# Autodesk Inventor assembly: Assembly_v1
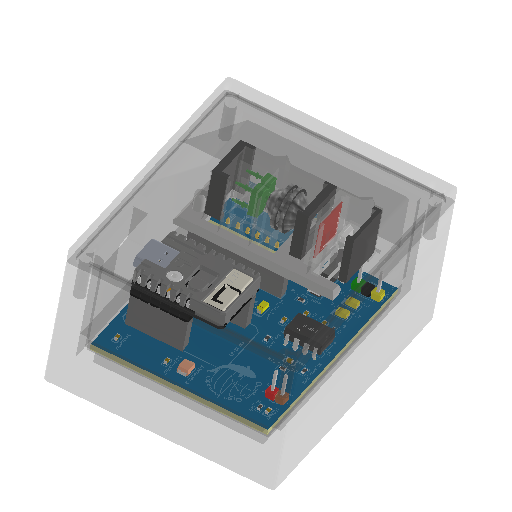
[picture p0: Inventor's stored thumbnail of the model, 512x512]
Saved by Autodesk Inventor 2026.1 (Build 301233020, 233B)
## iProperties
Created: 2026-01-21
Part Number: Assembly_v1
Document SubType Name: Assembly
Designer: samuel
Author: samuel
## Documents named in this file (18)
- E:\Fraunhofer\Design\Assembly_Box.iam
- E:\Fraunhofer\Design\Box_bottom_v2.ipt
- E:\Fraunhofer\Design\Parts\ads1015 ads1115 module type1\ads1015 ads1115 module type1\ads1015 ads1115 module type1.ipt
- E:\Fraunhofer\Design\Parts\USB C Male connector cable\USB C Male connector cable\USB C Male connector cable.ipt
- E:\Fraunhofer\Design\Assembly_NV__Optical_Modules.iam
- E:\Fraunhofer\Design\Parts\3D_PCB5_2026-02-13\3D_PCB5_2026-02-13\ESP32-S3~M5Stack StampS3 ~M5STAMP-S3.step~11hL.iam
- E:\Fraunhofer\Design\Parts\female-header-pins-2.snapshot.2\Female 6 Pin Header_\Female 6 Pin Header_\Female 6 Pin Header_.ipt
- E:\Fraunhofer\Design\Parts\female-header-pins-2.snapshot.2\Female 10 Pin Header\Female 10 Pin Header\Female 10 Pin Header.ipt
- E:\Fraunhofer\Design\Parts\female-header-pins-2.snapshot.2\Female 9 Pin Header\Female 9 Pin Header\Female 9 Pin Header.ipt
- E:\Fraunhofer\Design\Parts\3D_PCB5\3D_PCB5\3D_PCB5.iam
- E:\Fraunhofer\Design\Parts\2-54mm-male-pin-header-1.snapshot.3\Step\100mill Male Pin Header_10P_Y\100mill Male Pin Header_6P_Bk\100mill Male Pin Header_6P_Bk.ipt
- E:\Fraunhofer\Design\Parts\2-54mm-male-pin-header-1.snapshot.3\Step\100mill Male Pin Header_10P_Y\100mill Male Pin Header_9P_Bk\100mill Male Pin Header_9P_Bk.ipt
- E:\Fraunhofer\Design\Parts\2-54mm-male-pin-header-1.snapshot.3\Step\100mill Male Pin Header_2P_Bk\100mill Male Pin Header_2P_Bk\100mill Male Pin Header_2P_Bk.ipt
- E:\Fraunhofer\Design\Parts\2-54mm-male-pin-header-1.snapshot.3\Step\100mill Male Pin Header_3P_Bk\100mill Male Pin Header_3P_Bk\100mill Male Pin Header_3P_Bk.ipt
- E:\Fraunhofer\Design\Parts\dupont-jumper-wire-1.snapshot.3\Dupont Jumper Wire F-F\Dupont Jumper Wire F-F\Dupont Jumper Wire F-F.ipt
- E:\Fraunhofer\Design\Parts\dupont-jumper-wire-1.snapshot.3\Dupont Jumper Wire F-F\Dupont Jumper Wire F-F\Dupont Jumper Wire F-F - yellow.ipt
- E:\Fraunhofer\Design\Parts\dupont-jumper-wire-1.snapshot.3\Dupont Jumper Wire F-F\Dupont Jumper Wire F-F\Dupont Jumper Wire F-F - green.ipt
- E:\Fraunhofer\Design\Parts\dupont-jumper-wire-1.snapshot.3\Dupont Jumper Wire F-F\Dupont Jumper Wire F-F\Dupont Jumper Wire F-F - black.ipt
## Components (17 placed, 17 different names)
1. Box_bottom_v2:1 — Mate:10, Mate:13, Mate:21, Flush:19, Flush:20
2. ads1015 ads1115 module type1:1 — Flush:6, Flush:7, Mate:4
3. USB C Male connector cable:1 — Mate:19, Mate:20
4. Assembly_NV__Optical_Modules:1 [sub-assembly] — Flush:19, Flush:20
5. ESP32-S3~M5Stack StampS3 ~M5STAMP-S3.step~11hL:1 [sub-assembly] — Mate:8, Flush:8, Flush:9, Mate:9, Flush:10, Flush:11, Mate:19, Mate:20
6. 100mill Male Pin Header_6P_Bk:1 — Flush:12, Flush:13
7. 100mill Male Pin Header_9P_Bk:1 — Flush:14, Flush:15
8. Female 6 Pin Header_:1 — Mate:8, Flush:8, Flush:9, Mate:14, Mate:15, Mate:18, Flush:12, Flush:13
9. Female 10 Pin Header:1 — Flush:6, Flush:7, Mate:4, Mate:12, Mate:16, Mate:17
10. Female 9 Pin Header:1 — Mate:9, Flush:10, Flush:11, Flush:14, Flush:15
11. 3D_PCB5:1 [sub-assembly] — Mate:10, Mate:12, Mate:13, Mate:14, Mate:15, Mate:16, Mate:17, Mate:18, Mate:21, Mate:22, Flush:16, Mate:23, Flush:17
12. 100mill Male Pin Header_2P_Bk:1 — Mate:22, Flush:16, Flush:18, Mate:24, Flush:21, Flush:22, Flush:23, Mate:25
13. 100mill Male Pin Header_3P_Bk:1 — Mate:23, Flush:17, Flush:24, Flush:25, Flush:26, Mate:26, Flush:27, Mate:27
14. Dupont Jumper Wire F-F:1 — Flush:18, Mate:24, Flush:23
15. Dupont Jumper Wire F-F - yellow:1 — Flush:24, Flush:25, Mate:27
16. Dupont Jumper Wire F-F - green:1 — Flush:26, Mate:26, Flush:27
17. Dupont Jumper Wire F-F - black:1 — Flush:21, Flush:22, Mate:25
## Relationships (42: Flush 22, Mate 20)
- Flush:6: ads1015 ads1115 module type1:1 ↔ Female 10 Pin Header:1
- Flush:7: ads1015 ads1115 module type1:1 ↔ Female 10 Pin Header:1
- Mate:4: ads1015 ads1115 module type1:1 ↔ Female 10 Pin Header:1
- Mate:8 (2.5 mm): ESP32-S3~M5Stack StampS3 ~M5STAMP-S3.step~11hL:1 ↔ Female 6 Pin Header_:1
- Flush:8: ESP32-S3~M5Stack StampS3 ~M5STAMP-S3.step~11hL:1 ↔ Female 6 Pin Header_:1
- Flush:9 (0.6 mm): ESP32-S3~M5Stack StampS3 ~M5STAMP-S3.step~11hL:1 ↔ Female 6 Pin Header_:1
- Mate:9 (2.5 mm): ESP32-S3~M5Stack StampS3 ~M5STAMP-S3.step~11hL:1 ↔ Female 9 Pin Header:1
- Flush:10 (0.65 mm): ESP32-S3~M5Stack StampS3 ~M5STAMP-S3.step~11hL:1 ↔ Female 9 Pin Header:1
- Flush:11: ESP32-S3~M5Stack StampS3 ~M5STAMP-S3.step~11hL:1 ↔ Female 9 Pin Header:1
- Mate:10: Box_bottom_v2:1 ↔ 3D_PCB5:1
- Mate:12: Female 10 Pin Header:1 ↔ 3D_PCB5:1
- Mate:13: Box_bottom_v2:1 ↔ 3D_PCB5:1
- Mate:14: Female 6 Pin Header_:1 ↔ 3D_PCB5:1
- Mate:15 (-0.4 mm): Female 6 Pin Header_:1 ↔ 3D_PCB5:1
- Mate:16: Female 10 Pin Header:1 ↔ 3D_PCB5:1
- Mate:17: Female 10 Pin Header:1 ↔ 3D_PCB5:1
- Mate:18 (1.3 mm): Female 6 Pin Header_:1 ↔ 3D_PCB5:1
- Mate:19: USB C Male connector cable:1 ↔ ESP32-S3~M5Stack StampS3 ~M5STAMP-S3.step~11hL:1
- Mate:20: USB C Male connector cable:1 ↔ ESP32-S3~M5Stack StampS3 ~M5STAMP-S3.step~11hL:1
- Mate:21 (0.5 mm): Box_bottom_v2:1 ↔ 3D_PCB5:1
- Flush:12: 100mill Male Pin Header_6P_Bk:1 ↔ Female 6 Pin Header_:1
- Flush:13: 100mill Male Pin Header_6P_Bk:1 ↔ Female 6 Pin Header_:1
- Flush:14: 100mill Male Pin Header_9P_Bk:1 ↔ Female 9 Pin Header:1
- Flush:15: 100mill Male Pin Header_9P_Bk:1 ↔ Female 9 Pin Header:1
- Mate:22: 3D_PCB5:1 ↔ 100mill Male Pin Header_2P_Bk:1
- Flush:16 (1.2 mm): 3D_PCB5:1 ↔ 100mill Male Pin Header_2P_Bk:1
- Mate:23: 3D_PCB5:1 ↔ 100mill Male Pin Header_3P_Bk:1
- Flush:17 (1 mm): 3D_PCB5:1 ↔ 100mill Male Pin Header_3P_Bk:1
- Flush:18 (0.6 mm): 100mill Male Pin Header_2P_Bk:1 ↔ Dupont Jumper Wire F-F:1
- Mate:24: 100mill Male Pin Header_2P_Bk:1 ↔ Dupont Jumper Wire F-F:1
- Flush:19: Box_bottom_v2:1 ↔ Assembly_NV__Optical_Modules:1
- Flush:20: Box_bottom_v2:1 ↔ Assembly_NV__Optical_Modules:1
- Flush:21 (0.7 mm): 100mill Male Pin Header_2P_Bk:1 ↔ Dupont Jumper Wire F-F - black:1
- Flush:22 (0.7 mm): 100mill Male Pin Header_2P_Bk:1 ↔ Dupont Jumper Wire F-F - black:1
- Flush:23 (0.7 mm): 100mill Male Pin Header_2P_Bk:1 ↔ Dupont Jumper Wire F-F:1
- Mate:25: 100mill Male Pin Header_2P_Bk:1 ↔ Dupont Jumper Wire F-F - black:1
- Flush:24 (0.7 mm): 100mill Male Pin Header_3P_Bk:1 ↔ Dupont Jumper Wire F-F - yellow:1
- Flush:25 (0.6 mm): 100mill Male Pin Header_3P_Bk:1 ↔ Dupont Jumper Wire F-F - yellow:1
- Flush:26 (0.6 mm): 100mill Male Pin Header_3P_Bk:1 ↔ Dupont Jumper Wire F-F - green:1
- Mate:26: 100mill Male Pin Header_3P_Bk:1 ↔ Dupont Jumper Wire F-F - green:1
- Flush:27 (0.7 mm): 100mill Male Pin Header_3P_Bk:1 ↔ Dupont Jumper Wire F-F - green:1
- Mate:27: 100mill Male Pin Header_3P_Bk:1 ↔ Dupont Jumper Wire F-F - yellow:1
